# Autodesk Inventor assembly: Head Assemble
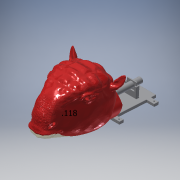
[picture p0: Inventor's stored thumbnail of the model, 180x180]
Saved by Autodesk Inventor 2019 (Build 230136000, 136)
## iProperties
Created: 2019-06-07
Part Number: Head Assemble
Document SubType Name: Assembly
Designer: Cole
Author: Cole
## Documents named in this file (8)
- G:\My Drive\Clubs\MTHS TSA\Animatronics 2019\Glyptodon\Glyptodon Work\Head\Head Assemble.iam
- G:\My Drive\Clubs\MTHS TSA\Animatronics 2019\Glyptodon\Glyptodon Work\Head\Head Workable With Mouth.ipt
- G:\My Drive\Clubs\MTHS TSA\Animatronics 2019\Glyptodon\Glyptodon Work\Head\Mouth.ipt
- G:\My Drive\Clubs\MTHS TSA\Animatronics 2019\Glyptodon\Glyptodon Work\Syringe Mounts\SyringeAttachment.ipt
- G:\My Drive\Clubs\MTHS TSA\Animatronics 2019\Glyptodon\Glyptodon Work\MudBox Exports\Better Syringe.iam
- G:\My Drive\Clubs\MTHS TSA\Animatronics 2019\Glyptodon\Glyptodon Work\Head\SyringeHeadLeverAttachmentNew.ipt
- G:\My Drive\Clubs\MTHS TSA\Animatronics 2019\Glyptodon - Nats\Glyptodon Work\Head\HeadBottom1.ipt
- G:\My Drive\Clubs\MTHS TSA\Animatronics 2019\To be reviewed\Reiden Copies\LeverArmMouth.ipt
## Components (9 placed, 7 different names)
1. Head Workable With Mouth:1 — Flush:1, Mate:1, Mate:2, Mate:3, Angle:1, Flush:2, Flush:3, Mate:20, Flush:10, Mate:28, Flush:11, Mate:29, Mate:33
2. Mouth:1 — Mate:1, Mate:2, Mate:33
3. SyringeAttachment:1 — Mate:15, Mate:25, Mate:26, Angle:4
4. SyringeAttachment:2 — Mate:21, Mate:22, Mate:23, Mate:24
5. Better Syringe:1 [sub-assembly] — Mate:15, Mate:16, Mate:17, Angle:3, Mate:23, Mate:26, Mate:27, Angle:4
6. SyringeHeadLeverAttachmentNew:1 — Mate:16, Mate:17, Angle:3, Flush:12, Mate:30, Mate:32
7. HeadBottom1:1 — Mate:20, Flush:10, Mate:21, Mate:22, Mate:24, Mate:25, Mate:27, Mate:28, Flush:11, Mate:29
8. LeverArmMouth:1 — Flush:12, Mate:31
9. LeverArmMouth:2 — Mate:30, Mate:31, Mate:32
## Relationships (29: Mate 20, Flush 6, Angle 3)
- Flush:1 (-298.45 mm): Head Workable With Mouth:1
- Mate:1 (0.5 mm): Head Workable With Mouth:1 ↔ Mouth:1
- Mate:2: Head Workable With Mouth:1 ↔ Mouth:1
- Mate:3: Head Workable With Mouth:1
- Angle:1 (0 deg): Head Workable With Mouth:1
- Flush:2 (21.844 mm): Head Workable With Mouth:1
- Flush:3: Head Workable With Mouth:1
- Mate:15: SyringeAttachment:1 ↔ Better Syringe:1
- Mate:16: Better Syringe:1 ↔ SyringeHeadLeverAttachmentNew:1
- Mate:17: Better Syringe:1 ↔ SyringeHeadLeverAttachmentNew:1
- Angle:3 (180 deg): Better Syringe:1 ↔ SyringeHeadLeverAttachmentNew:1
- Mate:20 (0.25 mm): Head Workable With Mouth:1 ↔ HeadBottom1:1
- Flush:10: Head Workable With Mouth:1 ↔ HeadBottom1:1
- Mate:21: SyringeAttachment:2 ↔ HeadBottom1:1
- Mate:22 (0.25 mm): SyringeAttachment:2 ↔ HeadBottom1:1
- Mate:23: SyringeAttachment:2 ↔ Better Syringe:1
- Mate:24: SyringeAttachment:2 ↔ HeadBottom1:1
- Mate:25: SyringeAttachment:1 ↔ HeadBottom1:1
- Mate:26: SyringeAttachment:1 ↔ Better Syringe:1
- Mate:27 (1 mm): Better Syringe:1 ↔ HeadBottom1:1
- Mate:28 (0.25 mm): Head Workable With Mouth:1 ↔ HeadBottom1:1
- Flush:11: Head Workable With Mouth:1 ↔ HeadBottom1:1
- Mate:29 (0.25 mm): Head Workable With Mouth:1 ↔ HeadBottom1:1
- Angle:4 (0 deg): SyringeAttachment:1 ↔ Better Syringe:1
- Flush:12: SyringeHeadLeverAttachmentNew:1 ↔ LeverArmMouth:1
- Mate:30: SyringeHeadLeverAttachmentNew:1 ↔ LeverArmMouth:2
- Mate:31: LeverArmMouth:1 ↔ LeverArmMouth:2
- Mate:32: SyringeHeadLeverAttachmentNew:1 ↔ LeverArmMouth:2
- Mate:33: Head Workable With Mouth:1 ↔ Mouth:1
